# Autodesk Inventor assembly: s-assy-frame-connector
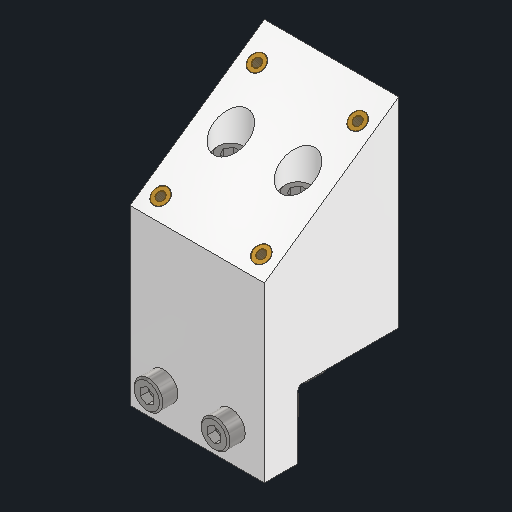
[picture p0: Inventor's stored thumbnail of the model, 512x512]
Saved by Autodesk Inventor 2022 (Build 260153000, 153)
## iProperties
Created: 2021-09-21
Part Number: s-assy-frame-connector
Document SubType Name: Assembly
Designer: yuto6
Mass: 104.335 g
Surface Area: 195.287 cm^2
Volume: 86.8438 cm^3
Density: 1.20141 g/cm^3
Author: yuto6
## Documents named in this file (6)
- C:\Users\yuta0\Desktop\catchrobo_shooter\s-assy-frame-connector.iam
- C:\Users\yuta0\Desktop\catchrobo_shooter\shooter_base2.ipt
- C:\Users\yuta0\Desktop\catchrobo_shooter\SB-305060.ipt
- C:\Users\yuta0\Desktop\catchrobo_shooter\CB5_40.ipt
- C:\Users\yuta0\Desktop\catchrobo_shooter\CB5-15.ipt
- C:\Users\yuta0\Desktop\catchrobo_shooter\HNTT5-5.ipt
## Components (13 placed, 5 different names)
1. shooter_base2:1 — メイト:7, フラッシュ:3, メイト:10, メイト:11, メイト:14, メイト:17, 角度:1, メイト:24, メイト:25, 角度:2
2. SB-305060:1 — メイト:7, フラッシュ:3
3. SB-305060:2
4. SB-305060:3
5. SB-305060:4
6. HNTT5-5:1 — メイト:22, 角度:1, メイト:25
7. CB5-15:1 — メイト:14, メイト:17, メイト:22
8. HNTT5-5:2 — メイト:23, メイト:24, 角度:2
9. CB5_40:1 — メイト:10, メイト:11, メイト:23
10. HNTT5-5:3
11. CB5-15:2
12. HNTT5-5:4
13. CB5_40:2
## Component patterns: (4 elements, first: SB-305060:1), (2 elements, first: HNTT5-5:1 + CB5-15:1 + HNTT5-5:2 + CB5_40:1)
## Relationships (12: Mate 9, Angle 2, Flush 1)
- メイト:7 [Mate]: shooter_base2:1 ↔ SB-305060:1
- フラッシュ:3 [Flush]: shooter_base2:1 ↔ SB-305060:1
- メイト:10 [Mate]: shooter_base2:1 ↔ CB5_40:1
- メイト:11 [Mate]: shooter_base2:1 ↔ CB5_40:1
- メイト:14 [Mate]: shooter_base2:1 ↔ CB5-15:1
- メイト:17 [Mate]: shooter_base2:1 ↔ CB5-15:1
- メイト:22 [Mate]: HNTT5-5:1 ↔ CB5-15:1
- 角度:1 [Angle] (0 deg): shooter_base2:1 ↔ HNTT5-5:1
- メイト:23 [Mate]: HNTT5-5:2 ↔ CB5_40:1
- メイト:24 [Mate] (2 mm): shooter_base2:1 ↔ HNTT5-5:2
- メイト:25 [Mate] (2 mm): shooter_base2:1 ↔ HNTT5-5:1
- 角度:2 [Angle] (0 deg): shooter_base2:1 ↔ HNTT5-5:2
